# Autodesk Inventor assembly: HS-225MG
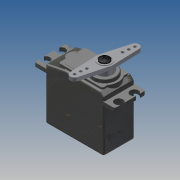
[picture p0: Inventor's stored thumbnail of the model, 180x180]
Saved by Autodesk Inventor 2012 SP2 (Build 160219200, 219)
## iProperties
Created: 2013-05-20
Part Number: HS-225MG
Document SubType Name: Assembly
Designer: Holger
Author: Holger
## Documents named in this file (4)
- M:\Modellbau\F550\Gimbal\HS-225MG.iam
- M:\Modellbau\F550\Gimbal\HS-225MG.ipt
- M:\Modellbau\F550\Gimbal\Ruderhorn.ipt
- C:\Users\Holger\Documents\Inventor\Content Center Files\R2011\de-DE\ISO 7049 - F-H(1)\ISO 7049 - ST2,9 x 6,5 - F - HDIN ISO.ipt
## Components (3 placed, 3 different names)
1. HS-225MG:1 — Einfügen:1
2. Ruderhorn:1 — Einfügen:1, Einfügen:2
3. DIN ISO 7049 - F-H ST2,9 x 6,5 - F - H:1 — Einfügen:2
## Relationships (2: Insert 2)
- Einfügen:1 [Insert]: HS-225MG:1 ↔ Ruderhorn:1
- Einfügen:2 [Insert] (-7.5 mm): Ruderhorn:1 ↔ DIN ISO 7049 - F-H ST2,9 x 6,5 - F - H:1
